# Autodesk Inventor assembly: Assembly
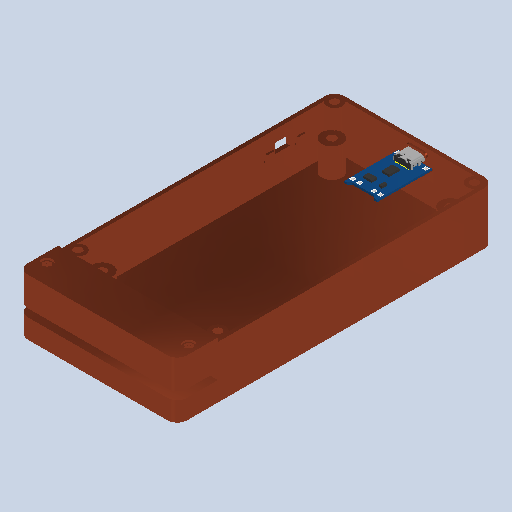
[picture p0: Inventor's stored thumbnail of the model, 512x512]
Saved by Autodesk Inventor 2026.2 (Build 302298000, 298)
## iProperties
Created: 2026-04-09
Part Number: Assembly
Document SubType Name: Assembly
Designer: Fork
Author: Fork
## Documents named in this file (9)
- D:\Smart\CAD\Assembly.iam
- D:\Smart\KiCad\step\model\model\model.ipt
- D:\Smart\CAD\basepcb.ipt
- D:\Smart\CAD\battery.ipt
- D:\Smart\KiCad\step\TCS34725 RGB sensor\TCS34725 RGB sensor\TCS34725 RGB sensor.ipt
- D:\Smart\KiCad\step\TP4056--3DModel-STEP-684600\TP4056--3DModel-STEP-684600\TP4056--3DModel-STEP-684600.ipt
- D:\Smart\CAD\toppcb.ipt
- D:\Smart\CAD\knob.ipt
- D:\Smart\CAD\colortop.ipt
## Components (9 placed, 8 different names)
1. model:1
2. basepcb:1 — Flush:1, Flush:3
3. battery:1
4. TCS34725 RGB sensor:1
5. TP4056--3DModel-STEP-684600:1
6. toppcb:1 — Flush:1, Flush:2
7. knob:1 — Flush:2
8. colortop:1 — Flush:3
9. basepcb:2
## Relationships (3: Flush 3)
- Flush:1: basepcb:1 ↔ toppcb:1
- Flush:2: toppcb:1 ↔ knob:1
- Flush:3: basepcb:1 ↔ colortop:1
